# Autodesk Inventor assembly: Swing_Arm_MIR
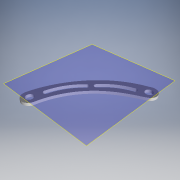
[picture p0: Inventor's stored thumbnail of the model, 180x180]
Saved by Autodesk Inventor 2016 (Build 200138000, 138)
## iProperties
Created: 2015-05-19
Part Number: Swing_Arm_MIR
Document SubType Name: Assembly
Designer: Yann
Author: Yann
## Documents named in this file (2)
- C:\Users\Yann\Documents\GitHub\BIKAIR_CAD\Source\Rear_Train\Swing_Arm_MIR.iam
- C:\Users\Yann\Documents\GitHub\BIKAIR_CAD\Source\Rear_Train\Profile_MIR.ipt
## Components (1 placed, 1 different names)
1. Profile_MIR:1 — Flush:1, Mate:1
## Relationships (2: Flush 1, Mate 1)
- Flush:1 (75 mm): Profile_MIR:1
- Mate:1: Profile_MIR:1
